# Autodesk Inventor assembly: Heatsink Holder
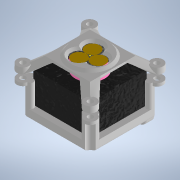
[picture p0: Inventor's stored thumbnail of the model, 180x180]
Saved by Autodesk Inventor 2021 (Build 250183000, 183)
## iProperties
Created: 2020-10-20
Part Number: Heatsink Holder
Document SubType Name: Assembly
Designer: VM
Author: VM
## Documents named in this file (5)
- \\vmware-host\Shared Folders\Documents\Projects Stuff\wakeuplamp\CAD\Heatsink Holder.iam
- \\vmware-host\Shared Folders\Documents\Projects Stuff\wakeuplamp\CAD\Heatsink.ipt
- \\vmware-host\Shared Folders\Documents\Projects Stuff\wakeuplamp\CAD\Back.ipt
- \\vmware-host\Shared Folders\Documents\Projects Stuff\wakeuplamp\CAD\LED and carclo.ipt
- \\vmware-host\Shared Folders\Documents\Projects Stuff\wakeuplamp\CAD\led holder.ipt
## Components (4 placed, 4 different names)
1. Heatsink:1 — Flush:1, Flush:2, Mate:1, Mate:2, Mate:3, Angle:1, Flush:3
2. Back:1 — Flush:1, Flush:2
3. LED and carclo:1 — Mate:1, Mate:2, Mate:3, Mate:4, Mate:5
4. led holder:1 — Mate:4, Mate:5, Angle:1, Flush:3
## Relationships (9: Mate 5, Flush 3, Angle 1)
- Flush:1: Heatsink:1 ↔ Back:1
- Flush:2: Heatsink:1 ↔ Back:1
- Mate:1: Heatsink:1 ↔ LED and carclo:1
- Mate:2 (-18.9 mm): Heatsink:1 ↔ LED and carclo:1
- Mate:3 (-18.65 mm): Heatsink:1 ↔ LED and carclo:1
- Mate:4: LED and carclo:1 ↔ led holder:1
- Mate:5: LED and carclo:1 ↔ led holder:1
- Angle:1 (0 deg): Heatsink:1 ↔ led holder:1
- Flush:3: Heatsink:1 ↔ led holder:1
